# Autodesk Inventor assembly: pistonMechanism-8-in
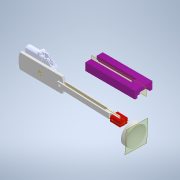
[picture p0: Inventor's stored thumbnail of the model, 180x180]
Saved by Autodesk Inventor 2020.2 (Build 242310000, 310)
## iProperties
Created: 2020-01-13
Part Number: pistonMechanism-8-in
Document SubType Name: Assembly
Designer: robst
Author: robst
## Documents named in this file (11)
- C:\git\CAD-Development\robSteele\2020BallTriggerMechanism\pistonMechanism-8-in.iam
- C:\git\CAD-Development\robSteele\2020BallTriggerMechanism\am-2235a Snow Blower Motor With Hex Shaft.iam
- C:\git\CAD-Development\robSteele\2020BallTriggerMechanism\am-2373 Snow Blower Motor Mount.ipt
- C:\git\CAD-Development\robSteele\2020BallTriggerMechanism\piston.ipt
- C:\git\CAD-Development\robSteele\2020BallTriggerMechanism\93365A162_HEAT-SET INSERTS FOR PLASTICS.ipt
- C:\git\CAD-Development\robSteele\2020BallTriggerMechanism\plateForBall.ipt
- C:\git\CAD-Development\robSteele\2020BallTriggerMechanism\plateRod.ipt
- C:\git\CAD-Development\robSteele\2020BallTriggerMechanism\driveForPiston-8-in.ipt
- C:\git\CAD-Development\robSteele\2020BallTriggerMechanism\connectingRodV02-8-in.ipt
- C:\git\CAD-Development\robSteele\2020BallTriggerMechanism\pistonHousing-8-in.ipt
- C:\git\CAD-Development\robSteele\2020BallTriggerMechanism\pistonHousingV03-8-in.ipt
## Components (12 placed, 10 different names)
1. driveForPiston-8-in:1 — Insert:3, Insert:10
2. am-2235a Snow Blower Motor With Hex Shaft:1 [sub-assembly] — Insert:1, Insert:2, Insert:3, Mate:1, Mate:3
3. am-2373 Snow Blower Motor Mount:1 — Insert:1, Insert:2
4. pistonHousing-8-in:1 — Mate:1, Mate:3, Flush:5
5. connectingRodV02-8-in:1 — Insert:10, Insert:11
6. piston:1 — Insert:11, Flush:5
7. 93365A162_HEAT-SET INSERTS FOR PLASTICS:1 — Insert:8
8. pistonHousing-8-in:2
9. plateForBall:1 — Insert:7, Insert:9
10. 93365A162_HEAT-SET INSERTS FOR PLASTICS:2 — Insert:7
11. plateRod:1 — Insert:8, Insert:9
12. pistonHousingV03-8-in:1
## Relationships (11: Insert 8, Mate 2, Flush 1)
- Insert:1: am-2235a Snow Blower Motor With Hex Shaft:1 ↔ am-2373 Snow Blower Motor Mount:1
- Insert:2: am-2235a Snow Blower Motor With Hex Shaft:1 ↔ am-2373 Snow Blower Motor Mount:1
- Insert:3: driveForPiston-8-in:1 ↔ am-2235a Snow Blower Motor With Hex Shaft:1
- Mate:1: am-2235a Snow Blower Motor With Hex Shaft:1 ↔ pistonHousing-8-in:1
- Mate:3 (165.1 mm): am-2235a Snow Blower Motor With Hex Shaft:1 ↔ pistonHousing-8-in:1
- Insert:7: plateForBall:1 ↔ 93365A162_HEAT-SET INSERTS FOR PLASTICS:2
- Insert:8 (-12.7 mm): 93365A162_HEAT-SET INSERTS FOR PLASTICS:1 ↔ plateRod:1
- Insert:9 (-12.7 mm): plateForBall:1 ↔ plateRod:1
- Insert:10: driveForPiston-8-in:1 ↔ connectingRodV02-8-in:1
- Insert:11: connectingRodV02-8-in:1 ↔ piston:1
- Flush:5: pistonHousing-8-in:1 ↔ piston:1
